# Autodesk Inventor assembly: assemlby
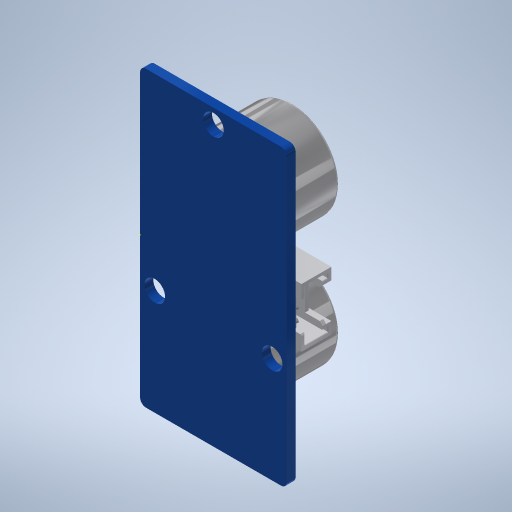
[picture p0: Inventor's stored thumbnail of the model, 512x512]
Saved by Autodesk Inventor 2023 (Build 270158000, 158)
## iProperties
Created: 2020-01-13
Part Number: assemlby
Material: Générique
Document SubType Name: Assembly
Designer: thoma
Author: thoma
## Documents named in this file (4)
- D:\Backup C\Documents\Inventor\PMLDCAPSTONE\Sensor Jarak\Grove_Ultrasonic_Sensor_V2.0.iam
- D:\Backup C\Documents\Inventor\PMLDCAPSTONE\Sensor Jarak\PCB.ipt
- D:\Backup C\Documents\Inventor\PMLDCAPSTONE\Sensor Jarak\sensor.ipt
- D:\Backup C\Documents\Inventor\PMLDCAPSTONE\Sensor Jarak\Grove_L_connector.ipt
## Components (4 placed, 3 different names)
1. PCB:1 — Affleurement:3, Placage:2, Affleurement:4, Placage:3, Placage:5, Affleurement:5, Placage:6
2. sensor:1 — Affleurement:3, Placage:3, Placage:4, Placage:5
3. sensor:2 — Placage:2, Affleurement:4, Placage:4
4. Grove_L_connector:1 — Affleurement:5, Placage:6
## Relationships (8: Mate 5, Flush 3)
- Affleurement:3 [Flush]: PCB:1 ↔ sensor:1
- Placage:2 [Mate]: PCB:1 ↔ sensor:2
- Affleurement:4 [Flush] (12.5 mm): PCB:1 ↔ sensor:2
- Placage:3 [Mate] (-12.5 mm): PCB:1 ↔ sensor:1
- Placage:4 [Mate] (22 mm): sensor:1 ↔ sensor:2
- Placage:5 [Mate] (-14 mm): PCB:1 ↔ sensor:1
- Affleurement:5 [Flush] (-1 mm): PCB:1 ↔ Grove_L_connector:1
- Placage:6 [Mate]: PCB:1 ↔ Grove_L_connector:1
